# Autodesk Inventor assembly: JB161410HC (1)
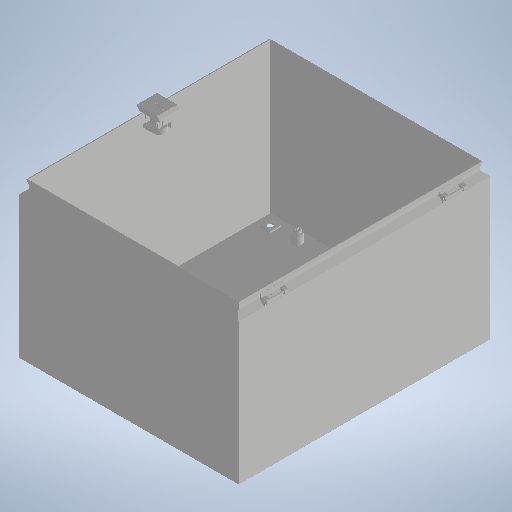
[picture p0: Inventor's stored thumbnail of the model, 512x512]
Saved by Autodesk Inventor 2025.2 (Build 292293000, 293)
## iProperties
Category: PARTsolutions
Company: RITTAL
Created: 2025-08-10
Part Number: JB161410HC (1)
Catalog Web Link: www.cadenas.de
Description: Hinged Cover-JB
Vendor: RITTAL
Document SubType Name: Assembly
Designer: psAdmin
Manufacturer: RITTAL
Mass: 8618.26 g
Surface Area: 16099.8 cm^2
Volume: 1280.15 cm^3
Density: 6.73223 g/cm^3
PSOL_IDENT_0: {$CADENAS_DATA/23d-libs/rittal/schaltschranksys/kleingeh/jb_parts/jb_asmtab.prj},201 {VTYP=3D},{STYP=
PSOL_IDENT_1: ASSTAB},{NB=JB161410HC (1)},{LINA=JB161410HC (1)},{NN=Hinged Cover},{DATE=20.08.2024 09:27:19},{GEOM
PSOL_IDENT_2: DATE=03.07.2019 13:23:22},{VERSION=},{LINEID=220},{WBVAR=DETAIL},{WBNUMERIC=DETAIL}  {NB=JB161410HC
PSOL_IDENT_3: (1)},{LINA=JB161410HC (1)},{KT=DUMMY},{PN=JB161410HC},{BEST=8018.127},{PN1=161410HC},{DETAIL=1},{H=1
PSOL_IDENT_4: 6},{B=14},{T=10},{W=19.0},{HM=400.00000},{BM=350.00000},{TM=250.00000},{ST=225.79000},{ETFT=8.19000}
PSOL_IDENT_5: ,{EPD=21.13000},{HHD=311.00000},{VHD=361.00000},{DMHD=284.40000},{EW=0.00000},{EH=0.00000},{MPX=225.
PSOL_IDENT_6: 00000},{MPY=361.00000},{MPN=4},{NOH=2},{MAT=CS},{MT=cs},{PPATH=jb_asmtpl.prj}
NB: JB161410HC (1)
NN: Hinged Cover
NT: JB
NBSYN: $PN. ($DETAIL.)
LINA: JB161410HC (1)
CATALOG: Rittal
PN: JB161410HC
BEST: 8018.127
DETAIL: High
H: 16
B: 14
T: 10
W: 19
SUPPLIER: RITTAL
ARTICLENO: JB161410HC (1)
BOMINFO: JB161410HC (1)
CREATOR: CADENAS GmbH
Title: JB161410HC (1)
Author: Cadenas PARTsolutions
Comments: JB
## Documents named in this file (9)
- C:\Users\cbast\OneDrive\Documents\GitHub\Smart-Pack-for-Advanced-Research-and-Control\variations\Camden\V0.2\Project Box CAD\RITTAL Enclosure\JB161410HC (1).iam
- C:\Users\cbast\OneDrive\Documents\GitHub\Smart-Pack-for-Advanced-Research-and-Control\variations\Camden\V0.2\Project Box CAD\RITTAL Enclosure\F161410HC1.ipt
- C:\Users\cbast\OneDrive\Documents\GitHub\Smart-Pack-for-Advanced-Research-and-Control\variations\Camden\V0.2\Project Box CAD\RITTAL Enclosure\JB_HINGE.ipt
- C:\Users\cbast\OneDrive\Documents\GitHub\Smart-Pack-for-Advanced-Research-and-Control\variations\Camden\V0.2\Project Box CAD\RITTAL Enclosure\jJBDOOR161410HC1.ipt
- C:\Users\cbast\OneDrive\Documents\GitHub\Smart-Pack-for-Advanced-Research-and-Control\variations\Camden\V0.2\Project Box CAD\RITTAL Enclosure\wm_one_door_lock_na.ipt
- C:\Users\cbast\OneDrive\Documents\GitHub\Smart-Pack-for-Advanced-Research-and-Control\variations\Camden\V0.2\Project Box CAD\RITTAL Enclosure\lock_insert_na.ipt
- C:\Users\cbast\OneDrive\Documents\GitHub\Smart-Pack-for-Advanced-Research-and-Control\variations\Camden\V0.2\Project Box CAD\RITTAL Enclosure\lock_washer_na.ipt
- C:\Users\cbast\OneDrive\Documents\GitHub\Smart-Pack-for-Advanced-Research-and-Control\variations\Camden\V0.2\Project Box CAD\RITTAL Enclosure\JBlock_plate.ipt
- C:\Users\cbast\OneDrive\Documents\GitHub\Smart-Pack-for-Advanced-Research-and-Control\variations\Camden\V0.2\Project Box CAD\RITTAL Enclosure\JBMP1614.ipt
## Components (9 placed, 8 different names)
1. F161410HC1:1 — s2_XY@1 <-> to_frame_XY@2, s2_Z@1 <-> to_frame_Z@2, s2_YZ@1 <-> to_frame_YZ@2, s1_XY@1 <-> to_frame_XY@3, s1_Z@1 <-> to_frame_Z@3, s1_YZ@1 <-> to_frame_YZ@3, to_plate_XY@1 <-> to_frame_XY@9, to_plate_Z@1 <-> to_frame_Z@9, to_plate_YZ@1 <-> to_frame_YZ@9
2. JB_HINGE:1 — s2_XY@1 <-> to_frame_XY@2, s2_Z@1 <-> to_frame_Z@2, s2_YZ@1 <-> to_frame_YZ@2
3. JB_HINGE:2 — s1_XY@1 <-> to_frame_XY@3, s1_Z@1 <-> to_frame_Z@3, s1_YZ@1 <-> to_frame_YZ@3, to_door_XY@3 <-> door_to_hinge_XY@4, to_door_Z@3 <-> door_to_hinge_Z@4, to_door_YZ@3 <-> door_to_hinge_YZ@4
4. jJBDOOR161410HC1:1 — to_door_XY@3 <-> door_to_hinge_XY@4, to_door_Z@3 <-> door_to_hinge_Z@4, to_door_YZ@3 <-> door_to_hinge_YZ@4, lock_XY@4 <-> lock_to_body_XY@5, lock_Z@4 <-> lock_to_body_Z@5, lock_YZ@4 <-> lock_to_body_YZ@5
5. wm_one_door_lock_na:1 — lock_XY@4 <-> lock_to_body_XY@5, lock_Z@4 <-> lock_to_body_Z@5, lock_YZ@4 <-> lock_to_body_YZ@5, insrt_to_lock_XY@5 <-> insert_to_lock_XY@6, insrt_to_lock_Z@5 <-> insert_to_lock_Z@6, insrt_to_lock_YZ@5 <-> insert_to_lock_YZ@6, washer_XY@5 <-> washer_to_insert_XY@7, washer_Z@5 <-> washer_to_insert_Z@7, washer_YZ@5 <-> washer_to_insert_YZ@7
6. lock_insert_na:1 — insrt_to_lock_XY@5 <-> insert_to_lock_XY@6, insrt_to_lock_Z@5 <-> insert_to_lock_Z@6, insrt_to_lock_YZ@5 <-> insert_to_lock_YZ@6
7. lock_washer_na:1 — washer_XY@5 <-> washer_to_insert_XY@7, washer_Z@5 <-> washer_to_insert_Z@7, washer_YZ@5 <-> washer_to_insert_YZ@7, washer_to_base_XY@7 <-> bottom_to_ins_XY@8, washer_to_base_Z@7 <-> bottom_to_ins_Z@8, washer_to_base_YZ@7 <-> bottom_to_ins_YZ@8
8. JBlock_plate:1 — washer_to_base_XY@7 <-> bottom_to_ins_XY@8, washer_to_base_Z@7 <-> bottom_to_ins_Z@8, washer_to_base_YZ@7 <-> bottom_to_ins_YZ@8
9. JBMP1614:1 — to_plate_XY@1 <-> to_frame_XY@9, to_plate_Z@1 <-> to_frame_Z@9, to_plate_YZ@1 <-> to_frame_YZ@9
## Relationships (24: Mate 9, Angle 8, Flush 7)
- s2_XY@1 <-> to_frame_XY@2 [Flush]: F161410HC1:1 ↔ JB_HINGE:1
- s2_Z@1 <-> to_frame_Z@2 [Mate]: F161410HC1:1 ↔ JB_HINGE:1
- s2_YZ@1 <-> to_frame_YZ@2 [Angle] (180 deg): F161410HC1:1 ↔ JB_HINGE:1
- s1_XY@1 <-> to_frame_XY@3 [Flush]: F161410HC1:1 ↔ JB_HINGE:2
- s1_Z@1 <-> to_frame_Z@3 [Mate]: F161410HC1:1 ↔ JB_HINGE:2
- s1_YZ@1 <-> to_frame_YZ@3 [Angle] (180 deg): F161410HC1:1 ↔ JB_HINGE:2
- to_door_XY@3 <-> door_to_hinge_XY@4 [Flush]: JB_HINGE:2 ↔ jJBDOOR161410HC1:1
- to_door_Z@3 <-> door_to_hinge_Z@4 [Mate]: JB_HINGE:2 ↔ jJBDOOR161410HC1:1
- to_door_YZ@3 <-> door_to_hinge_YZ@4 [Angle] (180 deg): JB_HINGE:2 ↔ jJBDOOR161410HC1:1
- lock_XY@4 <-> lock_to_body_XY@5 [Mate]: jJBDOOR161410HC1:1 ↔ wm_one_door_lock_na:1
- lock_Z@4 <-> lock_to_body_Z@5 [Mate]: jJBDOOR161410HC1:1 ↔ wm_one_door_lock_na:1
- lock_YZ@4 <-> lock_to_body_YZ@5 [Angle] (0 deg): jJBDOOR161410HC1:1 ↔ wm_one_door_lock_na:1
- insrt_to_lock_XY@5 <-> insert_to_lock_XY@6 [Flush]: wm_one_door_lock_na:1 ↔ lock_insert_na:1
- insrt_to_lock_Z@5 <-> insert_to_lock_Z@6 [Mate]: wm_one_door_lock_na:1 ↔ lock_insert_na:1
- insrt_to_lock_YZ@5 <-> insert_to_lock_YZ@6 [Angle] (0 deg): wm_one_door_lock_na:1 ↔ lock_insert_na:1
- washer_XY@5 <-> washer_to_insert_XY@7 [Flush]: wm_one_door_lock_na:1 ↔ lock_washer_na:1
- washer_Z@5 <-> washer_to_insert_Z@7 [Mate]: wm_one_door_lock_na:1 ↔ lock_washer_na:1
- washer_YZ@5 <-> washer_to_insert_YZ@7 [Angle] (90 deg): wm_one_door_lock_na:1 ↔ lock_washer_na:1
- washer_to_base_XY@7 <-> bottom_to_ins_XY@8 [Flush]: lock_washer_na:1 ↔ JBlock_plate:1
- washer_to_base_Z@7 <-> bottom_to_ins_Z@8 [Mate]: lock_washer_na:1 ↔ JBlock_plate:1
- washer_to_base_YZ@7 <-> bottom_to_ins_YZ@8 [Angle] (-90 deg): lock_washer_na:1 ↔ JBlock_plate:1
- to_plate_XY@1 <-> to_frame_XY@9 [Flush]: F161410HC1:1 ↔ JBMP1614:1
- to_plate_Z@1 <-> to_frame_Z@9 [Mate]: F161410HC1:1 ↔ JBMP1614:1
- to_plate_YZ@1 <-> to_frame_YZ@9 [Angle] (0 deg): F161410HC1:1 ↔ JBMP1614:1
